# Autodesk Inventor assembly: 000.001 - Ходовая часть
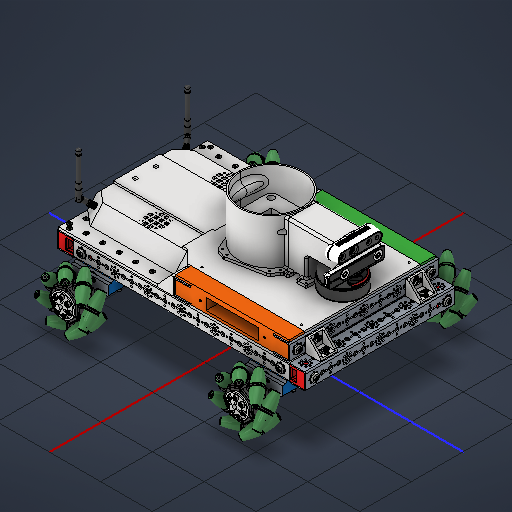
[picture p0: Inventor's stored thumbnail of the model, 512x512]
Saved by Autodesk Inventor 2025 (Build 290162000, 162)
## iProperties
Created: 2022-01-16
Part Number: 000.001 - Ходовая часть
Document SubType Name: Assembly
Designer: Петров Иван
Mass: 5535.1 g
Surface Area: 26163.7 cm^2
Volume: 4501.07 cm^3
Density: 1.22973 g/cm^3
Author: Петров Иван
## Documents named in this file (41)
- D:\Projects\OmniBot\design\000.001 - Ходовая часть.iam
- D:\Projects\OmniBot\design\standart_components\Tetrix\ftc-tetrix-kit-of-parts-1.snapshot.34\MAX Channels\416mm Channel.ipt
- D:\Projects\OmniBot\design\standart_components\Tetrix\Tetrix_Kit_FTC\tetrix_288mm_channel.ipt
- D:\Projects\OmniBot\design\000.001.001 - Уголок.ipt
- D:\Projects\OmniBot\design\000.002 - Крепеж мотора СБ.iam
- D:\Projects\OmniBot\design\000.001.002 - Днище.ipt
- D:\Projects\OmniBot\design\000.001.003 - Уголок.ipt
- D:\Projects\OmniBot\design\000.001.004 - Уголок.ipt
- D:\Projects\OmniBot\design\Content Center Files\R2022\ru-RU\BS 4183(4)\BS 4183 - M8 x 30(1) III.ipt
- D:\Projects\OmniBot\design\Content Center Files\R2022\ru-RU\ISO 4032(2)\ISO 4032 - M8 - ISO.ipt
- D:\Projects\OmniBot\design\Content Center Files\R2022\ru-RU\ISO 4762(2)\ISO 4762 - M4 x 35ISO.ipt
- D:\Projects\OmniBot\design\Content Center Files\R2022\ru-RU\ISO 4033(2)\ISO 4033 - M8 - ISO.ipt
- D:\Projects\OmniBot\design\Content Center Files\R2022\ru-RU\ISO 4032(2)\ISO 4032 - M4 - ISO.ipt
- D:\Projects\OmniBot\design\000.001.005 - Уголок.ipt
- D:\Projects\OmniBot\design\Content Center Files\R2022\ru-RU\BS 4183(4)\BS 4183 - M8 x 35(1) III.ipt
- D:\Projects\OmniBot\design\Content Center Files\R2022\ru-RU\ISO 7045  Z\ISO 7045 - M4 x 8_ - 4.8 - Z - ISO.ipt
- D:\Projects\OmniBot\design\000.003 - Крепление под XT60 мама.iam
- D:\Projects\OmniBot\design\000.004 - Крепление XT60 папа.iam
- D:\Projects\OmniBot\design\Content Center Files\ru-RU\ISO 7045(1)\DIN EN ISO 7045 - M4 x 12 - 4.8 - H.ipt
- D:\Projects\OmniBot\design\000.005 - Блок АКБ.iam
- D:\Projects\OmniBot\design\standart_components\OrangePi 5 Plus LTS\PI_MINI_PC_MAIN_PCB_ASM.iam
- D:\Projects\OmniBot\design\000.006 - Драйвер двигателя.iam
- D:\Projects\OmniBot\design\000.001.006 - Накладка.ipt
- D:\Projects\OmniBot\design\000.001.006 - Накладка зеркальный.ipt
- D:\Projects\OmniBot\design\Content Center Files\ru-RU\ISO 10642(1)\ISO 10642 - M4 x  8.ipt
- D:\Projects\OmniBot\design\standart_components\SMA_Connector_PART\SMA_Connector_PART.ipt
- D:\Projects\OmniBot\design\standart_components\wifi antenna\Antenna\Antenna.iam
- D:\Projects\OmniBot\design\Content Center Files\ru-RU\ISO 10642(1)\ISO 10642 - M4 x  12.ipt
- D:\Projects\OmniBot\design\000.006 - Драйвер двигателя зеркальный.iam
- D:\Projects\OmniBot\design\standart_components\CabelChannel\30x30mm\30x30mm.ipt
- D:\Projects\OmniBot\design\000.008 - Бортовой источник питания 5V СБ.iam
- D:\Projects\OmniBot\design\000.009 - Бортовой источник питания 3V3 СБ.iam
- D:\Projects\OmniBot\design\000.010 - Крышка.iam
- D:\Projects\OmniBot\design\000.001.007 - Короб.ipt
- D:\Projects\OmniBot\design\000.001.008 - Короб.ipt
- D:\Projects\OmniBot\design\standart_components\Mini Rocker 4-Pin Switch.ipt
- D:\Projects\OmniBot\design\standart_components\OrangePi 5 Plus LTS\OPI-5PLUS-PCBA.iam
- D:\Projects\OmniBot\design\000.001 - Ходовая часть_Упростить_1.ipt
- D:\Projects\OmniBot\design\for ros\ros_base_link.ipt
- D:\Projects\OmniBot\design\000.001 - Ходовая часть_Упростить_3.ipt
- D:\Projects\OmniBot\design\000.001 - Ходовая часть_Упростить_4.ipt
## Components (147 placed, 35 different names)
1. 000.001.001 - Уголок.ipt:1 — Совмещение:55, Совмещение:56, Совмещение:57, Совмещение:58, Совмещение:162, Совмещение:170
2. 000.001.001 - Уголок.ipt:2 — Совмещение:59, Совмещение:60, Совмещение:61, Совмещение:156, Совмещение:168
3. 000.001.001 - Уголок.ipt:3 — Совмещение:62, Совмещение:63, Совмещение:64, Совмещение:164, Совмещение:172
4. 000.001.001 - Уголок.ipt:4 — Совмещение:65, Совмещение:66, Совмещение:67, Совмещение:160, Совмещение:174
5. 000.001.002 - Днище.ipt:1 — Совмещение:88, Совмещение:90, Совмещение:91, Вставка:27, Вставка:28, Вставка:29, Вставка:30, Вставка:31, Вставка:32, Вставка:33, Вставка:34, Вставка:35, Вставка:36, Вставка:37, Вставка:38, Вставка:85, Вставка:86, Совмещение:350, Совмещение:401, Заподлицо:366, Совмещение:403, Заподлицо:368, Совмещение:404, Заподлицо:370, Заподлицо:371, Совмещение:407, Совмещение:410, Совмещение:427, Заподлицо:378, Заподлицо:380, Заподлицо:382, Заподлицо:385
6. 000.001.003 - Уголок.ipt:1 — Совмещение:109, Совмещение:110, Совмещение:111, Совмещение:158, Совмещение:419
7. 000.001.003 - Уголок.ipt:2 — Совмещение:112, Совмещение:113, Совмещение:114, Вставка:42, Совмещение:421
8. 000.001.003 - Уголок.ipt:3 — Совмещение:115, Совмещение:116, Совмещение:117, Вставка:41, Заподлицо:237, Совмещение:346, Совмещение:423, Совмещение:424
9. 000.001.003 - Уголок.ipt:4 — Совмещение:118, Совмещение:119, Совмещение:120, Совмещение:166
10. 000.001.004 - Уголок.ipt:1 — Совмещение:138, Совмещение:139, Вставка:43, Вставка:44, Вставка:45, Вставка:46, Вставка:47, Вставка:48
11. 000.001.004 - Уголок.ipt:2 — Совмещение:140, Совмещение:141, Совмещение:142, Вставка:49, Вставка:50, Вставка:51, Вставка:52, Вставка:53, Вставка:54
12. 000.001.005 - Уголок.ipt:1 — Совмещение:175, Совмещение:176, Совмещение:177, Вставка:39, Вставка:55, Вставка:56, Вставка:57, Заподлицо:365
13. 000.001.005 - Уголок.ipt:2 — Совмещение:178, Совмещение:179, Вставка:40, Вставка:58, Вставка:59, Вставка:60, Совмещение:357, Заподлицо:364, Совмещение:413
14. 000.002 - Крепеж мотора СБ.iam:1 [sub-assembly] — Совмещение:74, Совмещение:75, Совмещение:76, Касательность:1, Вставка:19, Вставка:20, Вставка:21, Вставка:22
15. 000.002 - Крепеж мотора СБ.iam:2 [sub-assembly] — Совмещение:77, Совмещение:79, Совмещение:152, Вставка:7, Вставка:8, Вставка:9, Вставка:10
16. 000.002 - Крепеж мотора СБ.iam:3 [sub-assembly] — Совмещение:80, Совмещение:82, Совмещение:154, Вставка:15, Вставка:16, Вставка:17, Вставка:18
17. 000.002 - Крепеж мотора СБ.iam:4 [sub-assembly] — Совмещение:83, Совмещение:84, Совмещение:153, Вставка:11, Вставка:12, Вставка:13, Вставка:14
18. 416mm Channel.ipt:1 — Совмещение:27, Совмещение:52, Заподлицо:1, Заподлицо:2, Совмещение:59, Совмещение:65, Совмещение:66, Совмещение:67, Совмещение:68, Совмещение:70, Совмещение:71, Совмещение:80, Совмещение:82, Совмещение:83, Совмещение:84, Совмещение:105, Совмещение:153, Совмещение:154, Вставка:25, Вставка:26, Совмещение:175, Совмещение:177, Совмещение:351, Совмещение:420
19. 416mm Channel.ipt:2 — Заподлицо:3, Заподлицо:4, Совмещение:53, Заподлицо:5, Заподлицо:6, Совмещение:54, Совмещение:55, Совмещение:56, Совмещение:57, Совмещение:62, Совмещение:69, Совмещение:74, Совмещение:76, Совмещение:77, Совмещение:79, Совмещение:88, Совмещение:91, Совмещение:104, Совмещение:152, Вставка:23, Вставка:24, Совмещение:179, Совмещение:358, Совмещение:408
20. tetrix_288mm_channel.ipt:1 — Совмещение:51, Заподлицо:5, Заподлицо:6, Совмещение:54, Совмещение:63, Совмещение:64, Совмещение:90, Вставка:5, Вставка:6, Совмещение:349, Совмещение:375
21. tetrix_288mm_channel.ipt:2 — Совмещение:52, Заподлицо:1, Заподлицо:2, Заподлицо:3, Заподлицо:4, Совмещение:53, Совмещение:58, Совмещение:60, Совмещение:61, Совмещение:75, Совмещение:138, Совмещение:139, Совмещение:140, Совмещение:141, Вставка:2, Вставка:3
22. tetrix_288mm_channel.ipt:3 — Совмещение:68, Совмещение:69, Совмещение:70, Совмещение:109, Совмещение:110, Совмещение:111, Совмещение:118, Совмещение:119, Совмещение:120, Совмещение:142, Вставка:1, Вставка:4, Угол:3, Заподлицо:238, Угол:7, Совмещение:402, Совмещение:415, Совмещение:417, Заподлицо:387
23. tetrix_288mm_channel.ipt:4 — Совмещение:71, Совмещение:104, Совмещение:105, Совмещение:112, Совмещение:113, Совмещение:114, Совмещение:115, Совмещение:116, Совмещение:117, Совмещение:176, Совмещение:178, Совмещение:343, Совмещение:344, Совмещение:345, Совмещение:347, Совмещение:376, Совмещение:411, Совмещение:418, Совмещение:422
24. 000.003 - Крепление под XT60 мама:1 [sub-assembly] — Совмещение:343, Совмещение:344, Совмещение:345, Совмещение:348, Угол:4, Совмещение:414
25. 000.004 - Крепление XT60 папа:1 [sub-assembly] — Заподлицо:237, Совмещение:346, Совмещение:347, Совмещение:348, Угол:4
26. DIN EN ISO 7045 H M4 x 12 - 4.8 - H:1 — Вставка:85
27. DIN EN ISO 7045 H M4 x 12 - 4.8 - H:2 — Вставка:86
28. 000.005 - Блок АКБ:1 [sub-assembly] — Совмещение:349, Совмещение:350, Совмещение:351, Угол:9
29. PI_MINI_PC_MAIN_PCB_ASM:1 [sub-assembly] — Заподлицо:238, Угол:7, Угол:8, Совмещение:409
30. 000.006 - Драйвер двигателя:1 [sub-assembly] — Совмещение:401, Заподлицо:366, Совмещение:402, Заподлицо:367, Заподлицо:372, Заподлицо:373
31. 000.006 - Драйвер двигателя:2 [sub-assembly] — Совмещение:403, Заподлицо:367, Заподлицо:368, Заподлицо:369
32. 000.001.006 - Накладка:1 — Совмещение:357, Совмещение:358, Заподлицо:364, Совмещение:359, Совмещение:360, Совмещение:361, Совмещение:362, Совмещение:363, Совмещение:364, Совмещение:365, Совмещение:366, Совмещение:379, Совмещение:380, Угол:5, Совмещение:385, Совмещение:386, Совмещение:387, Совмещение:388, Совмещение:389
33. 000.001.006 - Накладка зеркальный:1 — Совмещение:367, Совмещение:368, Совмещение:369, Совмещение:370, Совмещение:371, Совмещение:372, Совмещение:373, Совмещение:374, Заподлицо:365, Совмещение:375, Совмещение:376, Совмещение:377, Совмещение:378, Угол:6, Совмещение:390, Совмещение:391, Совмещение:392, Совмещение:393, Совмещение:394, Совмещение:412
34. SMA_Connector_PART:1 — Совмещение:377, Совмещение:378, Совмещение:382, Совмещение:383
35. SMA_Connector_PART:2 — Совмещение:379, Совмещение:380, Совмещение:381, Совмещение:384
36. Antenna:1 [sub-assembly] — Совмещение:381, Совмещение:384, Угол:5
37. Antenna:2 [sub-assembly] — Совмещение:382, Совмещение:383, Угол:6
38. 000.006 - Драйвер двигателя зеркальный:1 [sub-assembly] — Заподлицо:371, Заподлицо:372, Заподлицо:373
39. 000.006 - Драйвер двигателя зеркальный:2 [sub-assembly] — Совмещение:404, Заподлицо:369, Заподлицо:370
40. 30x30mm:2 — Совмещение:407, Угол:8, Совмещение:408, Совмещение:409, Совмещение:414
41. 000.008 - Бортовой источник питания СБ:1 [sub-assembly] — Совмещение:410, Угол:9, Совмещение:411, Совмещение:412, Заподлицо:375, Заподлицо:376
42. 000.009 - Бортовой источник питания 3V3 СБ:1 [sub-assembly] — Заподлицо:375, Заподлицо:376, Совмещение:413
43. 000.010 - Крышка:1 [sub-assembly] — Совмещение:415, Совмещение:417, Совмещение:418
44. 000.001.007 - Короб:1 — Совмещение:419, Совмещение:420, Совмещение:421, Совмещение:425, Совмещение:426, Заподлицо:377
45. 000.001.007 - Короб:2 — Совмещение:422, Совмещение:423, Совмещение:424
46. Mini Rocker 4-Pin Switch:1 — Совмещение:425, Совмещение:426, Заподлицо:377
47. 000.006 - Драйвер двигателя:3 [sub-assembly] — Заподлицо:379, Заподлицо:380, Заподлицо:383
48. 000.006 - Драйвер двигателя:4 [sub-assembly] — Совмещение:427, Заподлицо:378, Заподлицо:379, Заподлицо:381, Заподлицо:384, Заподлицо:386
49. 000.006 - Драйвер двигателя зеркальный:3 [sub-assembly] — Заподлицо:381, Заподлицо:382, Заподлицо:383
50. 000.006 - Драйвер двигателя зеркальный:4 [sub-assembly] — Заподлицо:384, Заподлицо:385, Заподлицо:386
51. OPI-5PLUS-PCBA:1 [sub-assembly] — Заподлицо:387
52. BS 4183 - M8 x 30(1) III.ipt:1 — Вставка:1, Совмещение:165
53. BS 4183 - M8 x 30(1) III.ipt:2 — Вставка:26, Совмещение:173
54. BS 4183 - M8 x 30(1) III.ipt:3 — Вставка:2, Совмещение:161
55. BS 4183 - M8 x 30(1) III.ipt:4 — Вставка:3, Совмещение:155
56. BS 4183 - M8 x 30(1) III.ipt:5 — Вставка:4, Совмещение:157
57. BS 4183 - M8 x 30(1) III.ipt:6 — Вставка:5, Совмещение:159
58. BS 4183 - M8 x 30(1) III.ipt:7 — Вставка:6, Совмещение:163
59. BS 4183 - M8 x 30(1) III.ipt:8 — Вставка:23, Совмещение:171
60. BS 4183 - M8 x 30(1) III.ipt:9 — Вставка:24, Совмещение:169
61. BS 4183 - M8 x 30(1) III.ipt:10 — Вставка:25, Совмещение:167
62. ISO 4032 - M4 - ISO.ipt:1 — Вставка:27
63. ISO 4032 - M4 - ISO.ipt:2 — Вставка:36
64. ISO 4032 - M4 - ISO.ipt:3 — Вставка:37
65. ISO 4032 - M4 - ISO.ipt:4 — Вставка:38
66. ISO 4032 - M4 - ISO.ipt:5 — Вставка:28
67. ISO 4032 - M4 - ISO.ipt:6 — Вставка:29
68. ISO 4032 - M4 - ISO.ipt:7 — Вставка:30
69. ISO 4032 - M4 - ISO.ipt:8 — Вставка:31
70. ISO 4032 - M4 - ISO.ipt:9 — Вставка:32
71. ISO 4032 - M4 - ISO.ipt:10 — Вставка:33
72. ISO 4032 - M4 - ISO.ipt:11 — Вставка:34
73. ISO 4032 - M4 - ISO.ipt:12 — Вставка:35
74. ISO 4032 - M8 - ISO.ipt:1 — Совмещение:155, Совмещение:156
75. ISO 4032 - M8 - ISO.ipt:2 — Совмещение:157, Совмещение:158
76. ISO 4032 - M8 - ISO.ipt:3 — Совмещение:159, Совмещение:160
77. ISO 4032 - M8 - ISO.ipt:4 — Совмещение:161, Совмещение:162
78. ISO 4032 - M8 - ISO.ipt:5 — Совмещение:163, Совмещение:164
79. ISO 4032 - M8 - ISO.ipt:6 — Совмещение:165, Совмещение:166
80. ISO 4033 - M8 - ISO.ipt:1 — Совмещение:167, Совмещение:168
81. ISO 4033 - M8 - ISO.ipt:2 — Совмещение:169, Совмещение:170
82. ISO 4033 - M8 - ISO.ipt:3 — Совмещение:171, Совмещение:172
83. ISO 4033 - M8 - ISO.ipt:4 — Совмещение:173, Совмещение:174
84. ISO 4762 - M4 x 35ISO.ipt:1 — Вставка:7
85. ISO 4762 - M4 x 35ISO.ipt:2 — Вставка:16
86. ISO 4762 - M4 x 35ISO.ipt:3 — Вставка:17
87. ISO 4762 - M4 x 35ISO.ipt:4 — Вставка:18
88. ISO 4762 - M4 x 35ISO.ipt:5 — Вставка:19
89. ISO 4762 - M4 x 35ISO.ipt:6 — Вставка:20
90. ISO 4762 - M4 x 35ISO.ipt:7 — Вставка:21
91. ISO 4762 - M4 x 35ISO.ipt:8 — Вставка:22
92. ISO 4762 - M4 x 35ISO.ipt:9 — Вставка:8
93. ISO 4762 - M4 x 35ISO.ipt:10 — Вставка:9
94. ISO 4762 - M4 x 35ISO.ipt:11 — Вставка:10
95. ISO 4762 - M4 x 35ISO.ipt:12 — Вставка:11
96. ISO 4762 - M4 x 35ISO.ipt:13 — Вставка:12
97. ISO 4762 - M4 x 35ISO.ipt:14 — Вставка:13
98. ISO 4762 - M4 x 35ISO.ipt:15 — Вставка:14
99. ISO 4762 - M4 x 35ISO.ipt:16 — Вставка:15
100. BS 4183 - M8 x 35(1) III.ipt:1 — Вставка:39
101. BS 4183 - M8 x 35(1) III.ipt:2 — Вставка:40
102. ISO 4032 - M8 - ISO.ipt:7 — Вставка:41
103. ISO 4032 - M8 - ISO.ipt:8 — Вставка:42
104. ISO 7045 - M4 x 8_ - 4.8 - Z - ISO.ipt:1 — Вставка:43
105. ISO 7045 - M4 x 8_ - 4.8 - Z - ISO.ipt:2 — Вставка:52
106. ISO 7045 - M4 x 8_ - 4.8 - Z - ISO.ipt:3 — Вставка:53
107. ISO 7045 - M4 x 8_ - 4.8 - Z - ISO.ipt:4 — Вставка:54
108. ISO 7045 - M4 x 8_ - 4.8 - Z - ISO.ipt:5 — Вставка:55
109. ISO 7045 - M4 x 8_ - 4.8 - Z - ISO.ipt:6 — Вставка:56
110. ISO 7045 - M4 x 8_ - 4.8 - Z - ISO.ipt:7 — Вставка:57
111. ISO 7045 - M4 x 8_ - 4.8 - Z - ISO.ipt:8 — Вставка:58
112. ISO 7045 - M4 x 8_ - 4.8 - Z - ISO.ipt:9 — Вставка:59
113. ISO 7045 - M4 x 8_ - 4.8 - Z - ISO.ipt:10 — Вставка:60
114. ISO 7045 - M4 x 8_ - 4.8 - Z - ISO.ipt:11 — Вставка:44
115. ISO 7045 - M4 x 8_ - 4.8 - Z - ISO.ipt:12 — Вставка:45
116. ISO 7045 - M4 x 8_ - 4.8 - Z - ISO.ipt:13 — Вставка:46
117. ISO 7045 - M4 x 8_ - 4.8 - Z - ISO.ipt:14 — Вставка:47
118. ISO 7045 - M4 x 8_ - 4.8 - Z - ISO.ipt:15 — Вставка:48
119. ISO 7045 - M4 x 8_ - 4.8 - Z - ISO.ipt:16 — Вставка:49
120. ISO 7045 - M4 x 8_ - 4.8 - Z - ISO.ipt:17 — Вставка:50
121. ISO 7045 - M4 x 8_ - 4.8 - Z - ISO.ipt:18 — Вставка:51
122. ISO 10642 M4x8:1 — Совмещение:359
123. ISO 10642 M4x8:2 — Совмещение:360
124. ISO 10642 M4x8:3 — Совмещение:361
125. ISO 10642 M4x8:4 — Совмещение:362
126. ISO 10642 M4x8:5 — Совмещение:363
127. ISO 10642 M4x8:6 — Совмещение:364
128. ISO 10642 M4x8:7 — Совмещение:365
129. ISO 10642 M4x8:8 — Совмещение:366
130. ISO 10642 M4x8:9 — Совмещение:367
131. ISO 10642 M4x8:10 — Совмещение:368
132. ISO 10642 M4x8:11 — Совмещение:369
133. ISO 10642 M4x8:12 — Совмещение:370
134. ISO 10642 M4x8:13 — Совмещение:371
135. ISO 10642 M4x8:14 — Совмещение:372
136. ISO 10642 M4x8:15 — Совмещение:373
137. ISO 10642 M4x8:16 — Совмещение:374
138. ISO 10642 M4x12:1 — Совмещение:385
139. ISO 10642 M4x12:2 — Совмещение:386
140. ISO 10642 M4x12:3 — Совмещение:387
141. ISO 10642 M4x12:4 — Совмещение:388
142. ISO 10642 M4x12:5 — Совмещение:389
143. ISO 10642 M4x12:6 — Совмещение:390
144. ISO 10642 M4x12:7 — Совмещение:391
145. ISO 10642 M4x12:8 — Совмещение:392
146. ISO 10642 M4x12:9 — Совмещение:393
147. ISO 10642 M4x12:10 — Совмещение:394
## Relationships (253: Mate 152, Insert 62, Flush 31, Angle 7, Tangent 1)
- Совмещение:27 [Mate]: 416mm Channel.ipt:1
- Совмещение:51 [Mate]: tetrix_288mm_channel.ipt:1
- Совмещение:52 [Mate]: 416mm Channel.ipt:1 ↔ tetrix_288mm_channel.ipt:2
- Заподлицо:1 [Flush]: 416mm Channel.ipt:1 ↔ tetrix_288mm_channel.ipt:2
- Заподлицо:2 [Flush]: 416mm Channel.ipt:1 ↔ tetrix_288mm_channel.ipt:2
- Заподлицо:3 [Flush]: 416mm Channel.ipt:2 ↔ tetrix_288mm_channel.ipt:2
- Заподлицо:4 [Flush]: 416mm Channel.ipt:2 ↔ tetrix_288mm_channel.ipt:2
- Совмещение:53 [Mate]: 416mm Channel.ipt:2 ↔ tetrix_288mm_channel.ipt:2
- Заподлицо:5 [Flush]: 416mm Channel.ipt:2 ↔ tetrix_288mm_channel.ipt:1
- Заподлицо:6 [Flush]: 416mm Channel.ipt:2 ↔ tetrix_288mm_channel.ipt:1
- Совмещение:54 [Mate]: 416mm Channel.ipt:2 ↔ tetrix_288mm_channel.ipt:1
- Совмещение:55 [Mate]: 000.001.001 - Уголок.ipt:1 ↔ 416mm Channel.ipt:2
- Совмещение:56 [Mate]: 000.001.001 - Уголок.ipt:1 ↔ 416mm Channel.ipt:2
- Совмещение:57 [Mate]: 000.001.001 - Уголок.ipt:1 ↔ 416mm Channel.ipt:2
- Совмещение:58 [Mate]: 000.001.001 - Уголок.ipt:1 ↔ tetrix_288mm_channel.ipt:2
- Совмещение:59 [Mate]: 000.001.001 - Уголок.ipt:2 ↔ 416mm Channel.ipt:1
- Совмещение:60 [Mate]: 000.001.001 - Уголок.ipt:2 ↔ tetrix_288mm_channel.ipt:2
- Совмещение:61 [Mate]: 000.001.001 - Уголок.ipt:2 ↔ tetrix_288mm_channel.ipt:2
- Совмещение:62 [Mate]: 000.001.001 - Уголок.ipt:3 ↔ 416mm Channel.ipt:2
- Совмещение:63 [Mate]: 000.001.001 - Уголок.ipt:3 ↔ tetrix_288mm_channel.ipt:1
- Совмещение:64 [Mate]: 000.001.001 - Уголок.ipt:3 ↔ tetrix_288mm_channel.ipt:1
- Совмещение:65 [Mate]: 000.001.001 - Уголок.ipt:4 ↔ 416mm Channel.ipt:1
- Совмещение:66 [Mate]: 000.001.001 - Уголок.ipt:4 ↔ 416mm Channel.ipt:1
- Совмещение:67 [Mate]: 000.001.001 - Уголок.ipt:4 ↔ 416mm Channel.ipt:1
- Совмещение:68 [Mate]: 416mm Channel.ipt:1 ↔ tetrix_288mm_channel.ipt:3
- Совмещение:69 [Mate]: 416mm Channel.ipt:2 ↔ tetrix_288mm_channel.ipt:3
- Совмещение:70 [Mate]: 416mm Channel.ipt:1 ↔ tetrix_288mm_channel.ipt:3
- Совмещение:71 [Mate]: 416mm Channel.ipt:1 ↔ tetrix_288mm_channel.ipt:4
- Совмещение:74 [Mate]: 000.002 - Крепеж мотора СБ.iam:1 ↔ 416mm Channel.ipt:2
- Совмещение:75 [Mate] (4 mm): 000.002 - Крепеж мотора СБ.iam:1 ↔ tetrix_288mm_channel.ipt:2
- Совмещение:76 [Mate]: 000.002 - Крепеж мотора СБ.iam:1 ↔ 416mm Channel.ipt:2
- Совмещение:77 [Mate]: 000.002 - Крепеж мотора СБ.iam:2 ↔ 416mm Channel.ipt:2
- Совмещение:79 [Mate]: 000.002 - Крепеж мотора СБ.iam:2 ↔ 416mm Channel.ipt:2
- Совмещение:80 [Mate]: 000.002 - Крепеж мотора СБ.iam:3 ↔ 416mm Channel.ipt:1
- Совмещение:82 [Mate]: 000.002 - Крепеж мотора СБ.iam:3 ↔ 416mm Channel.ipt:1
- Совмещение:83 [Mate]: 000.002 - Крепеж мотора СБ.iam:4 ↔ 416mm Channel.ipt:1
- Совмещение:84 [Mate]: 000.002 - Крепеж мотора СБ.iam:4 ↔ 416mm Channel.ipt:1
- Совмещение:88 [Mate]: 000.001.002 - Днище.ipt:1 ↔ 416mm Channel.ipt:2
- Совмещение:90 [Mate]: 000.001.002 - Днище.ipt:1 ↔ tetrix_288mm_channel.ipt:1
- Совмещение:91 [Mate]: 000.001.002 - Днище.ipt:1 ↔ 416mm Channel.ipt:2
- Совмещение:104 [Mate]: 416mm Channel.ipt:2 ↔ tetrix_288mm_channel.ipt:4
- Совмещение:105 [Mate]: 416mm Channel.ipt:1 ↔ tetrix_288mm_channel.ipt:4
- Совмещение:109 [Mate]: 000.001.003 - Уголок.ipt:1 ↔ tetrix_288mm_channel.ipt:3
- Совмещение:110 [Mate]: 000.001.003 - Уголок.ipt:1 ↔ tetrix_288mm_channel.ipt:3
- Совмещение:111 [Mate]: 000.001.003 - Уголок.ipt:1 ↔ tetrix_288mm_channel.ipt:3
- Совмещение:112 [Mate]: 000.001.003 - Уголок.ipt:2 ↔ tetrix_288mm_channel.ipt:4
- Совмещение:113 [Mate]: 000.001.003 - Уголок.ipt:2 ↔ tetrix_288mm_channel.ipt:4
- Совмещение:114 [Mate]: 000.001.003 - Уголок.ipt:2 ↔ tetrix_288mm_channel.ipt:4
- Совмещение:115 [Mate]: 000.001.003 - Уголок.ipt:3 ↔ tetrix_288mm_channel.ipt:4
- Совмещение:116 [Mate]: 000.001.003 - Уголок.ipt:3 ↔ tetrix_288mm_channel.ipt:4
- Совмещение:117 [Mate]: 000.001.003 - Уголок.ipt:3 ↔ tetrix_288mm_channel.ipt:4
- Совмещение:118 [Mate]: 000.001.003 - Уголок.ipt:4 ↔ tetrix_288mm_channel.ipt:3
- Совмещение:119 [Mate]: 000.001.003 - Уголок.ipt:4 ↔ tetrix_288mm_channel.ipt:3
- Совмещение:120 [Mate]: 000.001.003 - Уголок.ipt:4 ↔ tetrix_288mm_channel.ipt:3
- Совмещение:138 [Mate]: 000.001.004 - Уголок.ipt:1 ↔ tetrix_288mm_channel.ipt:2
- Совмещение:139 [Mate]: 000.001.004 - Уголок.ipt:1 ↔ tetrix_288mm_channel.ipt:2
- Совмещение:140 [Mate]: 000.001.004 - Уголок.ipt:2 ↔ tetrix_288mm_channel.ipt:2
- Совмещение:141 [Mate]: 000.001.004 - Уголок.ipt:2 ↔ tetrix_288mm_channel.ipt:2
- Совмещение:142 [Mate]: 000.001.004 - Уголок.ipt:2 ↔ tetrix_288mm_channel.ipt:3
- Касательность:1 [Tangent]: 000.002 - Крепеж мотора СБ.iam:1
- Совмещение:152 [Mate]: 000.002 - Крепеж мотора СБ.iam:2 ↔ 416mm Channel.ipt:2
- Совмещение:153 [Mate]: 000.002 - Крепеж мотора СБ.iam:4 ↔ 416mm Channel.ipt:1
- Совмещение:154 [Mate]: 000.002 - Крепеж мотора СБ.iam:3 ↔ 416mm Channel.ipt:1
- Вставка:1 [Insert]: tetrix_288mm_channel.ipt:3 ↔ BS 4183 - M8 x 30(1) III.ipt:1
- Вставка:2 [Insert]: tetrix_288mm_channel.ipt:2 ↔ BS 4183 - M8 x 30(1) III.ipt:3
- Вставка:3 [Insert]: tetrix_288mm_channel.ipt:2 ↔ BS 4183 - M8 x 30(1) III.ipt:4
- Вставка:4 [Insert]: tetrix_288mm_channel.ipt:3 ↔ BS 4183 - M8 x 30(1) III.ipt:5
- Вставка:5 [Insert]: tetrix_288mm_channel.ipt:1 ↔ BS 4183 - M8 x 30(1) III.ipt:6
- Вставка:6 [Insert]: tetrix_288mm_channel.ipt:1 ↔ BS 4183 - M8 x 30(1) III.ipt:7
- Совмещение:155 [Mate]: BS 4183 - M8 x 30(1) III.ipt:4 ↔ ISO 4032 - M8 - ISO.ipt:1
- Совмещение:156 [Mate]: 000.001.001 - Уголок.ipt:2 ↔ ISO 4032 - M8 - ISO.ipt:1
- Совмещение:157 [Mate]: BS 4183 - M8 x 30(1) III.ipt:5 ↔ ISO 4032 - M8 - ISO.ipt:2
- Совмещение:158 [Mate]: 000.001.003 - Уголок.ipt:1 ↔ ISO 4032 - M8 - ISO.ipt:2
- Совмещение:159 [Mate]: BS 4183 - M8 x 30(1) III.ipt:6 ↔ ISO 4032 - M8 - ISO.ipt:3
- Совмещение:160 [Mate]: 000.001.001 - Уголок.ipt:4 ↔ ISO 4032 - M8 - ISO.ipt:3
- Совмещение:161 [Mate]: BS 4183 - M8 x 30(1) III.ipt:3 ↔ ISO 4032 - M8 - ISO.ipt:4
- Совмещение:162 [Mate]: 000.001.001 - Уголок.ipt:1 ↔ ISO 4032 - M8 - ISO.ipt:4
- Совмещение:163 [Mate]: BS 4183 - M8 x 30(1) III.ipt:7 ↔ ISO 4032 - M8 - ISO.ipt:5
- Совмещение:164 [Mate]: 000.001.001 - Уголок.ipt:3 ↔ ISO 4032 - M8 - ISO.ipt:5
- Совмещение:165 [Mate]: BS 4183 - M8 x 30(1) III.ipt:1 ↔ ISO 4032 - M8 - ISO.ipt:6
- Совмещение:166 [Mate]: 000.001.003 - Уголок.ipt:4 ↔ ISO 4032 - M8 - ISO.ipt:6
- Вставка:7 [Insert]: 000.002 - Крепеж мотора СБ.iam:2 ↔ ISO 4762 - M4 x 35ISO.ipt:1
- Вставка:8 [Insert]: 000.002 - Крепеж мотора СБ.iam:2 ↔ ISO 4762 - M4 x 35ISO.ipt:9
- Вставка:9 [Insert]: 000.002 - Крепеж мотора СБ.iam:2 ↔ ISO 4762 - M4 x 35ISO.ipt:10
- Вставка:10 [Insert]: 000.002 - Крепеж мотора СБ.iam:2 ↔ ISO 4762 - M4 x 35ISO.ipt:11
- Вставка:11 [Insert]: 000.002 - Крепеж мотора СБ.iam:4 ↔ ISO 4762 - M4 x 35ISO.ipt:12
- Вставка:12 [Insert]: 000.002 - Крепеж мотора СБ.iam:4 ↔ ISO 4762 - M4 x 35ISO.ipt:13
- Вставка:13 [Insert]: 000.002 - Крепеж мотора СБ.iam:4 ↔ ISO 4762 - M4 x 35ISO.ipt:14
- Вставка:14 [Insert]: 000.002 - Крепеж мотора СБ.iam:4 ↔ ISO 4762 - M4 x 35ISO.ipt:15
- Вставка:15 [Insert]: 000.002 - Крепеж мотора СБ.iam:3 ↔ ISO 4762 - M4 x 35ISO.ipt:16
- Вставка:16 [Insert]: 000.002 - Крепеж мотора СБ.iam:3 ↔ ISO 4762 - M4 x 35ISO.ipt:2
- Вставка:17 [Insert]: 000.002 - Крепеж мотора СБ.iam:3 ↔ ISO 4762 - M4 x 35ISO.ipt:3
- Вставка:18 [Insert]: 000.002 - Крепеж мотора СБ.iam:3 ↔ ISO 4762 - M4 x 35ISO.ipt:4
- Вставка:19 [Insert]: 000.002 - Крепеж мотора СБ.iam:1 ↔ ISO 4762 - M4 x 35ISO.ipt:5
- Вставка:20 [Insert]: 000.002 - Крепеж мотора СБ.iam:1 ↔ ISO 4762 - M4 x 35ISO.ipt:6
- Вставка:21 [Insert]: 000.002 - Крепеж мотора СБ.iam:1 ↔ ISO 4762 - M4 x 35ISO.ipt:7
- Вставка:22 [Insert]: 000.002 - Крепеж мотора СБ.iam:1 ↔ ISO 4762 - M4 x 35ISO.ipt:8
- Вставка:23 [Insert]: 416mm Channel.ipt:2 ↔ BS 4183 - M8 x 30(1) III.ipt:8
- Вставка:24 [Insert]: 416mm Channel.ipt:2 ↔ BS 4183 - M8 x 30(1) III.ipt:9
- Вставка:25 [Insert]: 416mm Channel.ipt:1 ↔ BS 4183 - M8 x 30(1) III.ipt:10
- Вставка:26 [Insert]: 416mm Channel.ipt:1 ↔ BS 4183 - M8 x 30(1) III.ipt:2
- Совмещение:167 [Mate]: BS 4183 - M8 x 30(1) III.ipt:10 ↔ ISO 4033 - M8 - ISO.ipt:1
- Совмещение:168 [Mate]: 000.001.001 - Уголок.ipt:2 ↔ ISO 4033 - M8 - ISO.ipt:1
- Совмещение:169 [Mate]: BS 4183 - M8 x 30(1) III.ipt:9 ↔ ISO 4033 - M8 - ISO.ipt:2
- Совмещение:170 [Mate]: 000.001.001 - Уголок.ipt:1 ↔ ISO 4033 - M8 - ISO.ipt:2
- Совмещение:171 [Mate]: BS 4183 - M8 x 30(1) III.ipt:8 ↔ ISO 4033 - M8 - ISO.ipt:3
- Совмещение:172 [Mate]: 000.001.001 - Уголок.ipt:3 ↔ ISO 4033 - M8 - ISO.ipt:3
- Совмещение:173 [Mate]: BS 4183 - M8 x 30(1) III.ipt:2 ↔ ISO 4033 - M8 - ISO.ipt:4
- Совмещение:174 [Mate]: 000.001.001 - Уголок.ipt:4 ↔ ISO 4033 - M8 - ISO.ipt:4
- Вставка:27 [Insert]: 000.001.002 - Днище.ipt:1 ↔ ISO 4032 - M4 - ISO.ipt:1
- Вставка:28 [Insert]: 000.001.002 - Днище.ipt:1 ↔ ISO 4032 - M4 - ISO.ipt:5
- Вставка:29 [Insert]: 000.001.002 - Днище.ipt:1 ↔ ISO 4032 - M4 - ISO.ipt:6
- Вставка:30 [Insert]: 000.001.002 - Днище.ipt:1 ↔ ISO 4032 - M4 - ISO.ipt:7
- Вставка:31 [Insert]: 000.001.002 - Днище.ipt:1 ↔ ISO 4032 - M4 - ISO.ipt:8
- Вставка:32 [Insert]: 000.001.002 - Днище.ipt:1 ↔ ISO 4032 - M4 - ISO.ipt:9
- Вставка:33 [Insert]: 000.001.002 - Днище.ipt:1 ↔ ISO 4032 - M4 - ISO.ipt:10
- Вставка:34 [Insert]: 000.001.002 - Днище.ipt:1 ↔ ISO 4032 - M4 - ISO.ipt:11
- Вставка:35 [Insert]: 000.001.002 - Днище.ipt:1 ↔ ISO 4032 - M4 - ISO.ipt:12
- Вставка:36 [Insert]: 000.001.002 - Днище.ipt:1 ↔ ISO 4032 - M4 - ISO.ipt:2
- Вставка:37 [Insert]: 000.001.002 - Днище.ipt:1 ↔ ISO 4032 - M4 - ISO.ipt:3
- Вставка:38 [Insert]: 000.001.002 - Днище.ipt:1 ↔ ISO 4032 - M4 - ISO.ipt:4
- Совмещение:175 [Mate]: 000.001.005 - Уголок.ipt:1 ↔ 416mm Channel.ipt:1
- Совмещение:176 [Mate]: 000.001.005 - Уголок.ipt:1 ↔ tetrix_288mm_channel.ipt:4
- Совмещение:177 [Mate]: 000.001.005 - Уголок.ipt:1 ↔ 416mm Channel.ipt:1
- Совмещение:178 [Mate]: 000.001.005 - Уголок.ipt:2 ↔ tetrix_288mm_channel.ipt:4
- Совмещение:179 [Mate]: 000.001.005 - Уголок.ipt:2 ↔ 416mm Channel.ipt:2
- Вставка:39 [Insert]: 000.001.005 - Уголок.ipt:1 ↔ BS 4183 - M8 x 35(1) III.ipt:1
- Вставка:40 [Insert]: 000.001.005 - Уголок.ipt:2 ↔ BS 4183 - M8 x 35(1) III.ipt:2
- Вставка:41 [Insert]: 000.001.003 - Уголок.ipt:3 ↔ ISO 4032 - M8 - ISO.ipt:7
- Вставка:42 [Insert]: 000.001.003 - Уголок.ipt:2 ↔ ISO 4032 - M8 - ISO.ipt:8
- Вставка:43 [Insert]: 000.001.004 - Уголок.ipt:1 ↔ ISO 7045 - M4 x 8_ - 4.8 - Z - ISO.ipt:1
- Вставка:44 [Insert]: 000.001.004 - Уголок.ipt:1 ↔ ISO 7045 - M4 x 8_ - 4.8 - Z - ISO.ipt:11
- Вставка:45 [Insert]: 000.001.004 - Уголок.ipt:1 ↔ ISO 7045 - M4 x 8_ - 4.8 - Z - ISO.ipt:12
- Вставка:46 [Insert]: 000.001.004 - Уголок.ipt:1 ↔ ISO 7045 - M4 x 8_ - 4.8 - Z - ISO.ipt:13
- Вставка:47 [Insert]: 000.001.004 - Уголок.ipt:1 ↔ ISO 7045 - M4 x 8_ - 4.8 - Z - ISO.ipt:14
- Вставка:48 [Insert]: 000.001.004 - Уголок.ipt:1 ↔ ISO 7045 - M4 x 8_ - 4.8 - Z - ISO.ipt:15
- Вставка:49 [Insert]: 000.001.004 - Уголок.ipt:2 ↔ ISO 7045 - M4 x 8_ - 4.8 - Z - ISO.ipt:16
- Вставка:50 [Insert]: 000.001.004 - Уголок.ipt:2 ↔ ISO 7045 - M4 x 8_ - 4.8 - Z - ISO.ipt:17
- Вставка:51 [Insert]: 000.001.004 - Уголок.ipt:2 ↔ ISO 7045 - M4 x 8_ - 4.8 - Z - ISO.ipt:18
- Вставка:52 [Insert]: 000.001.004 - Уголок.ipt:2 ↔ ISO 7045 - M4 x 8_ - 4.8 - Z - ISO.ipt:2
- Вставка:53 [Insert]: 000.001.004 - Уголок.ipt:2 ↔ ISO 7045 - M4 x 8_ - 4.8 - Z - ISO.ipt:3
- Вставка:54 [Insert]: 000.001.004 - Уголок.ipt:2 ↔ ISO 7045 - M4 x 8_ - 4.8 - Z - ISO.ipt:4
- Вставка:55 [Insert]: 000.001.005 - Уголок.ipt:1 ↔ ISO 7045 - M4 x 8_ - 4.8 - Z - ISO.ipt:5
- Вставка:56 [Insert]: 000.001.005 - Уголок.ipt:1 ↔ ISO 7045 - M4 x 8_ - 4.8 - Z - ISO.ipt:6
- Вставка:57 [Insert]: 000.001.005 - Уголок.ipt:1 ↔ ISO 7045 - M4 x 8_ - 4.8 - Z - ISO.ipt:7
- Вставка:58 [Insert]: 000.001.005 - Уголок.ipt:2 ↔ ISO 7045 - M4 x 8_ - 4.8 - Z - ISO.ipt:8
- Вставка:59 [Insert]: 000.001.005 - Уголок.ipt:2 ↔ ISO 7045 - M4 x 8_ - 4.8 - Z - ISO.ipt:9
- Вставка:60 [Insert]: 000.001.005 - Уголок.ipt:2 ↔ ISO 7045 - M4 x 8_ - 4.8 - Z - ISO.ipt:10
- Угол:3 [Angle] (0 deg): tetrix_288mm_channel.ipt:3
- Совмещение:343 [Mate]: tetrix_288mm_channel.ipt:4 ↔ 000.003 - Крепление под XT60 мама:1
- Совмещение:344 [Mate]: tetrix_288mm_channel.ipt:4 ↔ 000.003 - Крепление под XT60 мама:1
- Совмещение:345 [Mate]: tetrix_288mm_channel.ipt:4 ↔ 000.003 - Крепление под XT60 мама:1
- Заподлицо:237 [Flush]: 000.001.003 - Уголок.ipt:3 ↔ 000.004 - Крепление XT60 папа:1
- Совмещение:346 [Mate]: 000.001.003 - Уголок.ipt:3 ↔ 000.004 - Крепление XT60 папа:1
- Совмещение:347 [Mate]: tetrix_288mm_channel.ipt:4 ↔ 000.004 - Крепление XT60 папа:1
- Совмещение:348 [Mate]: 000.003 - Крепление под XT60 мама:1 ↔ 000.004 - Крепление XT60 папа:1
- Угол:4 [Angle] (0 deg): 000.003 - Крепление под XT60 мама:1 ↔ 000.004 - Крепление XT60 папа:1
- Вставка:85 [Insert]: 000.001.002 - Днище.ipt:1 ↔ DIN EN ISO 7045 H M4 x 12 - 4.8 - H:1
- Вставка:86 [Insert]: 000.001.002 - Днище.ipt:1 ↔ DIN EN ISO 7045 H M4 x 12 - 4.8 - H:2
- Совмещение:349 [Mate]: tetrix_288mm_channel.ipt:1 ↔ 000.005 - Блок АКБ:1
- Совмещение:350 [Mate]: 000.001.002 - Днище.ipt:1 ↔ 000.005 - Блок АКБ:1
- Совмещение:351 [Mate] (77 mm): 416mm Channel.ipt:1 ↔ 000.005 - Блок АКБ:1
- Заподлицо:238 [Flush]: tetrix_288mm_channel.ipt:3 ↔ PI_MINI_PC_MAIN_PCB_ASM:1
- Совмещение:357 [Mate]: 000.001.005 - Уголок.ipt:2 ↔ 000.001.006 - Накладка:1
- Совмещение:358 [Mate]: 416mm Channel.ipt:2 ↔ 000.001.006 - Накладка:1
- Заподлицо:364 [Flush]: 000.001.005 - Уголок.ipt:2 ↔ 000.001.006 - Накладка:1
- Совмещение:359 [Mate]: 000.001.006 - Накладка:1 ↔ ISO 10642 M4x8:1
- Совмещение:360 [Mate]: 000.001.006 - Накладка:1 ↔ ISO 10642 M4x8:2
- Совмещение:361 [Mate]: 000.001.006 - Накладка:1 ↔ ISO 10642 M4x8:3
- Совмещение:362 [Mate]: 000.001.006 - Накладка:1 ↔ ISO 10642 M4x8:4
- Совмещение:363 [Mate]: 000.001.006 - Накладка:1 ↔ ISO 10642 M4x8:5
- Совмещение:364 [Mate]: 000.001.006 - Накладка:1 ↔ ISO 10642 M4x8:6
- Совмещение:365 [Mate]: 000.001.006 - Накладка:1 ↔ ISO 10642 M4x8:7
- Совмещение:366 [Mate]: 000.001.006 - Накладка:1 ↔ ISO 10642 M4x8:8
- Совмещение:367 [Mate]: 000.001.006 - Накладка зеркальный:1 ↔ ISO 10642 M4x8:9
- Совмещение:368 [Mate]: 000.001.006 - Накладка зеркальный:1 ↔ ISO 10642 M4x8:10
- Совмещение:369 [Mate]: 000.001.006 - Накладка зеркальный:1 ↔ ISO 10642 M4x8:11
- Совмещение:370 [Mate]: 000.001.006 - Накладка зеркальный:1 ↔ ISO 10642 M4x8:12
- Совмещение:371 [Mate]: 000.001.006 - Накладка зеркальный:1 ↔ ISO 10642 M4x8:13
- Совмещение:372 [Mate]: 000.001.006 - Накладка зеркальный:1 ↔ ISO 10642 M4x8:14
- Совмещение:373 [Mate]: 000.001.006 - Накладка зеркальный:1 ↔ ISO 10642 M4x8:15
- Совмещение:374 [Mate]: 000.001.006 - Накладка зеркальный:1 ↔ ISO 10642 M4x8:16
- Заподлицо:365 [Flush]: 000.001.005 - Уголок.ipt:1 ↔ 000.001.006 - Накладка зеркальный:1
- Совмещение:375 [Mate]: tetrix_288mm_channel.ipt:1 ↔ 000.001.006 - Накладка зеркальный:1
- Совмещение:376 [Mate]: tetrix_288mm_channel.ipt:4 ↔ 000.001.006 - Накладка зеркальный:1
- Совмещение:377 [Mate]: 000.001.006 - Накладка зеркальный:1 ↔ SMA_Connector_PART:1
- Совмещение:378 [Mate]: 000.001.006 - Накладка зеркальный:1 ↔ SMA_Connector_PART:1
- Совмещение:379 [Mate]: 000.001.006 - Накладка:1 ↔ SMA_Connector_PART:2
- Совмещение:380 [Mate]: 000.001.006 - Накладка:1 ↔ SMA_Connector_PART:2
- Совмещение:381 [Mate]: SMA_Connector_PART:2 ↔ Antenna:1
- Совмещение:382 [Mate]: SMA_Connector_PART:1 ↔ Antenna:2
- Совмещение:383 [Mate]: SMA_Connector_PART:1 ↔ Antenna:2
- Совмещение:384 [Mate]: SMA_Connector_PART:2 ↔ Antenna:1
- Угол:5 [Angle] (180 deg): 000.001.006 - Накладка:1 ↔ Antenna:1
- Угол:6 [Angle] (180 deg): 000.001.006 - Накладка зеркальный:1 ↔ Antenna:2
- Совмещение:385 [Mate]: 000.001.006 - Накладка:1 ↔ ISO 10642 M4x12:1
- Совмещение:386 [Mate]: 000.001.006 - Накладка:1 ↔ ISO 10642 M4x12:2
- Совмещение:387 [Mate]: 000.001.006 - Накладка:1 ↔ ISO 10642 M4x12:3
- Совмещение:388 [Mate]: 000.001.006 - Накладка:1 ↔ ISO 10642 M4x12:4
- Совмещение:389 [Mate]: 000.001.006 - Накладка:1 ↔ ISO 10642 M4x12:5
- Совмещение:390 [Mate]: 000.001.006 - Накладка зеркальный:1 ↔ ISO 10642 M4x12:6
- Совмещение:391 [Mate]: 000.001.006 - Накладка зеркальный:1 ↔ ISO 10642 M4x12:7
- Совмещение:392 [Mate]: 000.001.006 - Накладка зеркальный:1 ↔ ISO 10642 M4x12:8
- Совмещение:393 [Mate]: 000.001.006 - Накладка зеркальный:1 ↔ ISO 10642 M4x12:9
- Совмещение:394 [Mate]: 000.001.006 - Накладка зеркальный:1 ↔ ISO 10642 M4x12:10
- Угол:7 [Angle] (-90 deg): tetrix_288mm_channel.ipt:3 ↔ PI_MINI_PC_MAIN_PCB_ASM:1
- Совмещение:401 [Mate] (5 mm): 000.001.002 - Днище.ipt:1 ↔ 000.006 - Драйвер двигателя:1
- Заподлицо:366 [Flush] (5 mm): 000.001.002 - Днище.ipt:1 ↔ 000.006 - Драйвер двигателя:1
- Совмещение:402 [Mate]: tetrix_288mm_channel.ipt:3 ↔ 000.006 - Драйвер двигателя:1
- Совмещение:403 [Mate] (13 mm): 000.001.002 - Днище.ipt:1 ↔ 000.006 - Драйвер двигателя:2
- Заподлицо:367 [Flush]: 000.006 - Драйвер двигателя:1 ↔ 000.006 - Драйвер двигателя:2
- Заподлицо:368 [Flush] (-5 mm): 000.001.002 - Днище.ipt:1 ↔ 000.006 - Драйвер двигателя:2
- Совмещение:404 [Mate] (5 mm): 000.001.002 - Днище.ipt:1 ↔ 000.006 - Драйвер двигателя зеркальный:2
- Заподлицо:369 [Flush]: 000.006 - Драйвер двигателя:2 ↔ 000.006 - Драйвер двигателя зеркальный:2
- Заподлицо:370 [Flush] (5 mm): 000.001.002 - Днище.ipt:1 ↔ 000.006 - Драйвер двигателя зеркальный:2
- Заподлицо:371 [Flush] (5 mm): 000.001.002 - Днище.ipt:1 ↔ 000.006 - Драйвер двигателя зеркальный:1
- Заподлицо:372 [Flush]: 000.006 - Драйвер двигателя:1 ↔ 000.006 - Драйвер двигателя зеркальный:1
- Заподлицо:373 [Flush]: 000.006 - Драйвер двигателя:1 ↔ 000.006 - Драйвер двигателя зеркальный:1
- Совмещение:407 [Mate]: 000.001.002 - Днище.ipt:1 ↔ 30x30mm:2
- Угол:8 [Angle] (0 deg): PI_MINI_PC_MAIN_PCB_ASM:1 ↔ 30x30mm:2
- Совмещение:408 [Mate] (0.5 mm): 416mm Channel.ipt:2 ↔ 30x30mm:2
- Совмещение:409 [Mate] (3 mm): PI_MINI_PC_MAIN_PCB_ASM:1 ↔ 30x30mm:2
- Совмещение:410 [Mate] (15 mm): 000.001.002 - Днище.ipt:1 ↔ 000.008 - Бортовой источник питания СБ:1
- Угол:9 [Angle] (180 deg): 000.005 - Блок АКБ:1 ↔ 000.008 - Бортовой источник питания СБ:1
- Совмещение:411 [Mate] (10 mm): tetrix_288mm_channel.ipt:4 ↔ 000.008 - Бортовой источник питания СБ:1
- Совмещение:412 [Mate] (5 mm): 000.001.006 - Накладка зеркальный:1 ↔ 000.008 - Бортовой источник питания СБ:1
- Заподлицо:375 [Flush]: 000.008 - Бортовой источник питания СБ:1 ↔ 000.009 - Бортовой источник питания 3V3 СБ:1
- Заподлицо:376 [Flush]: 000.008 - Бортовой источник питания СБ:1 ↔ 000.009 - Бортовой источник питания 3V3 СБ:1
- Совмещение:413 [Mate] (15 mm): 000.001.005 - Уголок.ipt:2 ↔ 000.009 - Бортовой источник питания 3V3 СБ:1
- Совмещение:414 [Mate] (3 mm): 000.003 - Крепление под XT60 мама:1 ↔ 30x30mm:2
- Совмещение:415 [Mate]: tetrix_288mm_channel.ipt:3 ↔ 000.010 - Крышка:1
- Совмещение:417 [Mate]: tetrix_288mm_channel.ipt:3 ↔ 000.010 - Крышка:1
- Совмещение:418 [Mate]: tetrix_288mm_channel.ipt:4 ↔ 000.010 - Крышка:1
- Совмещение:419 [Mate]: 000.001.003 - Уголок.ipt:1 ↔ 000.001.007 - Короб:1
- Совмещение:420 [Mate]: 416mm Channel.ipt:1 ↔ 000.001.007 - Короб:1
- Совмещение:421 [Mate]: 000.001.003 - Уголок.ipt:2 ↔ 000.001.007 - Короб:1
- Совмещение:422 [Mate]: tetrix_288mm_channel.ipt:4 ↔ 000.001.007 - Короб:2
- Совмещение:423 [Mate]: 000.001.003 - Уголок.ipt:3 ↔ 000.001.007 - Короб:2
- Совмещение:424 [Mate]: 000.001.003 - Уголок.ipt:3 ↔ 000.001.007 - Короб:2
- Совмещение:425 [Mate]: 000.001.007 - Короб:1 ↔ Mini Rocker 4-Pin Switch:1
- Совмещение:426 [Mate]: 000.001.007 - Короб:1 ↔ Mini Rocker 4-Pin Switch:1
- Заподлицо:377 [Flush] (11 mm): 000.001.007 - Короб:1 ↔ Mini Rocker 4-Pin Switch:1
- Совмещение:427 [Mate] (5 mm): 000.001.002 - Днище.ipt:1 ↔ 000.006 - Драйвер двигателя:4
- Заподлицо:378 [Flush]: 000.001.002 - Днище.ipt:1 ↔ 000.006 - Драйвер двигателя:4
- Заподлицо:379 [Flush]: 000.006 - Драйвер двигателя:3 ↔ 000.006 - Драйвер двигателя:4
- Заподлицо:380 [Flush]: 000.001.002 - Днище.ipt:1 ↔ 000.006 - Драйвер двигателя:3
- Заподлицо:381 [Flush]: 000.006 - Драйвер двигателя:4 ↔ 000.006 - Драйвер двигателя зеркальный:3
- Заподлицо:382 [Flush]: 000.001.002 - Днище.ipt:1 ↔ 000.006 - Драйвер двигателя зеркальный:3
- Заподлицо:383 [Flush]: 000.006 - Драйвер двигателя:3 ↔ 000.006 - Драйвер двигателя зеркальный:3
- Заподлицо:384 [Flush]: 000.006 - Драйвер двигателя:4 ↔ 000.006 - Драйвер двигателя зеркальный:4
- Заподлицо:385 [Flush]: 000.001.002 - Днище.ipt:1 ↔ 000.006 - Драйвер двигателя зеркальный:4
- Заподлицо:386 [Flush]: 000.006 - Драйвер двигателя:4 ↔ 000.006 - Драйвер двигателя зеркальный:4
- Заподлицо:387 [Flush]: tetrix_288mm_channel.ipt:3 ↔ OPI-5PLUS-PCBA:1
